# Autodesk Inventor assembly: segment1
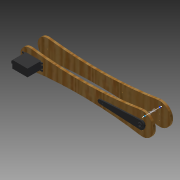
[picture p0: Inventor's stored thumbnail of the model, 180x180]
Saved by Autodesk Inventor 2013 (Build 170138000, 138)
## iProperties
Created: 2014-10-09
Part Number: segment1
Document SubType Name: Assembly
Designer: Masta
Author: Masta
## Documents named in this file (5)
- D:\DrOctopus\3D model\segment1.iam
- D:\DrOctopus\3D model\segment1a.ipt
- D:\DrOctopus\3D model\servo 13kg BMS-630MG.ipt
- D:\DrOctopus\3D model\segment1b.ipt
- D:\DrOctopus\3D model\servo arm TGY-S8166M long.ipt
## Components (4 placed, 4 different names)
1. segment1a:1 — Mate:1, Insert:1, Insert:2, Tangent:1, Insert:3, Tangent:2
2. servo 13kg BMS-630MG:1 — Mate:1, Insert:1
3. segment1b:1 — Insert:2, Tangent:1
4. servo arm TGY-S8166M long:1 — Insert:3, Tangent:2
## Relationships (6: Insert 3, Tangent 2, Mate 1)
- Mate:1: segment1a:1 ↔ servo 13kg BMS-630MG:1
- Insert:1 (1.7 mm): segment1a:1 ↔ servo 13kg BMS-630MG:1
- Insert:2 (40 mm): segment1a:1 ↔ segment1b:1
- Tangent:1: segment1a:1 ↔ segment1b:1
- Insert:3: segment1a:1 ↔ servo arm TGY-S8166M long:1
- Tangent:2: segment1a:1 ↔ servo arm TGY-S8166M long:1
